# Autodesk Inventor assembly: intake assembly
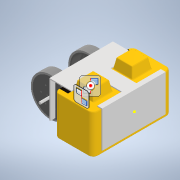
[picture p0: Inventor's stored thumbnail of the model, 180x180]
Saved by Autodesk Inventor 2020 (Build 240168000, 168)
## iProperties
Created: 2019-10-18
Part Number: intake assembly
Document SubType Name: Assembly
Designer: tdmp4
Author: tdmp4
## Documents named in this file (7)
- C:\Users\tdmp4\OneDrive\Documents\GitHub\CAD-2020\Intake\intake assembly.iam
- C:\Users\tdmp4\OneDrive\Documents\GitHub\CAD-2020\Intake\intakeCover.ipt
- C:\Users\tdmp4\OneDrive\Documents\GitHub\CAD-2020\ServoCity\585440.ipt
- C:\Users\tdmp4\OneDrive\Documents\GitHub\CAD-2020\ServoCity\535198.ipt
- C:\Users\tdmp4\OneDrive\Documents\GitHub\CAD-2020\ServoCity\634084.ipt
- C:\Users\tdmp4\OneDrive\Documents\GitHub\CAD-2020\Intake\intakeStealthSub.iam
- C:\Users\tdmp4\OneDrive\Documents\GitHub\CAD-2020\1x2 Block v2 Auto Real Decal.ipt
## Components (8 placed, 6 different names)
1. intakeCover:1 — Mate:1, Mate:2, Mate:3, Mate:13, Mate:14
2. 585440:1 — Mate:1, Mate:2, Mate:3, Mate:4, Mate:5, Mate:6, Mate:7, Flush:1
3. 535198:1 — Mate:4, Mate:5, Mate:11
4. 535198:2 — Mate:6, Mate:7, Mate:8, Mate:10
5. 634084:1 — Mate:8, Flush:1, Mate:9, Mate:12
6. intakeStealthSub:1 [sub-assembly] — Mate:9, Mate:10
7. intakeStealthSub:2 [sub-assembly] — Mate:11, Mate:12
8. 1x2 Block v2 Auto Real Decal:1 — Mate:13, Mate:14
## Relationships (15: Mate 14, Flush 1)
- Mate:1: intakeCover:1 ↔ 585440:1
- Mate:2: intakeCover:1 ↔ 585440:1
- Mate:3: intakeCover:1 ↔ 585440:1
- Mate:4: 585440:1 ↔ 535198:1
- Mate:5: 585440:1 ↔ 535198:1
- Mate:6: 585440:1 ↔ 535198:2
- Mate:7: 585440:1 ↔ 535198:2
- Mate:8: 535198:2 ↔ 634084:1
- Flush:1 (-69.85 mm): 585440:1 ↔ 634084:1
- Mate:9: 634084:1 ↔ intakeStealthSub:1
- Mate:10: 535198:2 ↔ intakeStealthSub:1
- Mate:11: 535198:1 ↔ intakeStealthSub:2
- Mate:12: 634084:1 ↔ intakeStealthSub:2
- Mate:13: intakeCover:1 ↔ 1x2 Block v2 Auto Real Decal:1
- Mate:14: intakeCover:1 ↔ 1x2 Block v2 Auto Real Decal:1
